# Autodesk Inventor assembly: bottom_assembly
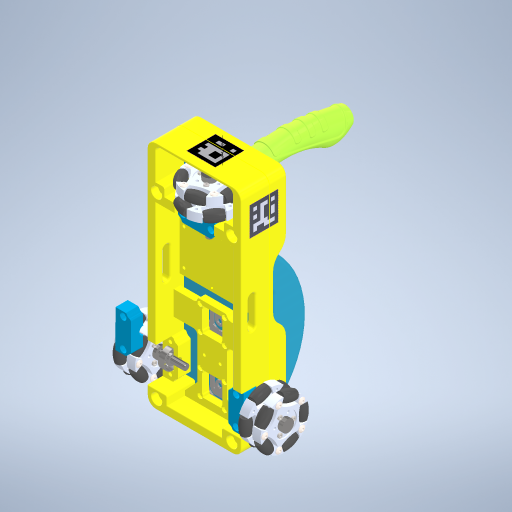
[picture p0: Inventor's stored thumbnail of the model, 512x512]
Saved by Autodesk Inventor 2024 (Build 280153000, 153)
## iProperties
Created: 2023-09-04
Part Number: bottom_assembly
Document SubType Name: Assembly
Designer: Pintu
Author: Pintu
## Documents named in this file (11)
- D:\CMC\my_inventor\ArmBo_v2\bottom_assembly.iam
- D:\CMC\my_inventor\ArmBo_v2\bottom_chassis_extended.ipt
- D:\CMC\my_inventor\ArmBo_v2\bearing_holder_bottom.ipt
- D:\CMC\my_inventor\ArmBo_v2\Shaft2.ipt
- D:\CMC\my_inventor\ArmBo_v2\support\WheelAsm\WheelAsm.iam
- D:\CMC\my_inventor\ArmBo_v2\bottom_assembly\Design Accelerator\Bearing2.iam
- D:\CMC\my_inventor\ArmBo_v2\spuare_load_cell.ipt
- D:\CMC\my_inventor\ArmBo_v2\pcb_dummy.ipt
- D:\CMC\my_inventor\ArmBo_v2\hand_rest_gamestick.ipt
- D:\CMC\my_inventor\ArmBo_v2\HOLDERS\flight_stick.ipt
- D:\CMC\my_inventor\ArmBo_v2\HOLDERS\handgrip_regular.ipt
## Components (18 placed, 10 different names)
1. bottom_chassis_extended:1 — Mate:1, Mate:2, Mate:6, Mate:7, Mate:8, Mate:9, Mate:11, Mate:12, Mate:13, Mate:18, Mate:19, Mate:20, Mate:21, Mate:22, Mate:23, Mate:24, Mate:25, Mate:26
2. bearing_holder_bottom:1
3. bearing_holder_bottom:2 — Mate:11
4. Shaft:1 — Mate:2, Mate:3, Mate:5
5. Shaft:2 — Mate:1, Mate:4
6. WheelAsm:1 [sub-assembly] — Mate:3
7. WheelAsm:2 [sub-assembly] — Mate:4
8. Bearing:1 [sub-assembly] — Mate:5, Mate:6, Mate:7
9. Bearing:2 [sub-assembly] — Mate:8, Mate:9
10. bearing_holder_bottom:3 — Mate:13
11. Shaft:3 — Mate:12, Mate:14
12. WheelAsm:3 [sub-assembly] — Mate:14
13. spuare_load_cell:1 — Mate:18, Mate:19
14. spuare_load_cell:2 — Mate:20, Mate:21
15. pcb_dummy:1 — Mate:22, Mate:23
16. hand_rest_gamestick:1 — Mate:24, Mate:25, Mate:26, Mate:27
17. flight_stick:1
18. handgrip_regular:1 — Mate:27
## Relationships (23: Mate 23)
- Mate:1: bottom_chassis_extended:1 ↔ Shaft:2
- Mate:2: bottom_chassis_extended:1 ↔ Shaft:1
- Mate:3: Shaft:1 ↔ WheelAsm:1
- Mate:4: Shaft:2 ↔ WheelAsm:2
- Mate:5: Shaft:1 ↔ Bearing:1
- Mate:6: bottom_chassis_extended:1 ↔ Bearing:1
- Mate:7: bottom_chassis_extended:1 ↔ Bearing:1
- Mate:8: bottom_chassis_extended:1 ↔ Bearing:2
- Mate:9: bottom_chassis_extended:1 ↔ Bearing:2
- Mate:11: bottom_chassis_extended:1 ↔ bearing_holder_bottom:2
- Mate:12: bottom_chassis_extended:1 ↔ Shaft:3
- Mate:13: bottom_chassis_extended:1 ↔ bearing_holder_bottom:3
- Mate:14: Shaft:3 ↔ WheelAsm:3
- Mate:18: bottom_chassis_extended:1 ↔ spuare_load_cell:1
- Mate:19: bottom_chassis_extended:1 ↔ spuare_load_cell:1
- Mate:20: bottom_chassis_extended:1 ↔ spuare_load_cell:2
- Mate:21: bottom_chassis_extended:1 ↔ spuare_load_cell:2
- Mate:22: bottom_chassis_extended:1 ↔ pcb_dummy:1
- Mate:23: bottom_chassis_extended:1 ↔ pcb_dummy:1
- Mate:24: bottom_chassis_extended:1 ↔ hand_rest_gamestick:1
- Mate:25 (2 mm): bottom_chassis_extended:1 ↔ hand_rest_gamestick:1
- Mate:26 (2 mm): bottom_chassis_extended:1 ↔ hand_rest_gamestick:1
- Mate:27 (1 mm): hand_rest_gamestick:1 ↔ handgrip_regular:1
